# Autodesk Inventor assembly: Assembly1
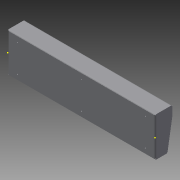
[picture p0: Inventor's stored thumbnail of the model, 180x180]
Saved by Autodesk Inventor 2015 (Build 190159000, 159)
## iProperties
Created: 2015-09-21
Part Number: Assembly1
Document SubType Name: Assembly
Designer: Komp
Author: Komp
## Documents named in this file (3)
- D:\obudowka projekcik\Assembly1.iam
- D:\obudowka projekcik\obodowka.ipt
- D:\obudowka projekcik\obodowka_cz_2.ipt
## Components (2 placed, 2 different names)
1. obodowka:1 — Mate:1, Mate:2
2. obodowka_cz_2:1 — Mate:1, Mate:2
## Relationships (2: Mate 2)
- Mate:1: obodowka:1 ↔ obodowka_cz_2:1
- Mate:2: obodowka:1 ↔ obodowka_cz_2:1
